# Autodesk Inventor assembly: hip_link2
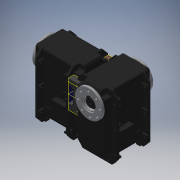
[picture p0: Inventor's stored thumbnail of the model, 180x180]
Saved by Autodesk Inventor 2018 (Build 220112000, 112)
## iProperties
Created: 2018-11-28
Part Number: hip_link2
Document SubType Name: Assembly
Designer: bitbots
Author: bitbots
## Documents named in this file (4)
- C:\Users\bitbots\Desktop\bitbots_hardware\wolfgang\assembly\legs\hip_link2.iam
- C:\Users\bitbots\Desktop\bitbots_hardware\wolfgang\assembly\motors\MX106\MX-106_with_bearing_MIR.iam
- C:\Users\bitbots\Desktop\bitbots_hardware\wolfgang\assembly\legs\motor_connector_MIR.ipt
- C:\Users\bitbots\Desktop\bitbots_hardware\wolfgang\assembly\motors\MX106\MX-106_with_horn_MIR.iam
## Components (4 placed, 3 different names)
1. MX-106_with_bearing_MIR:1 [sub-assembly]
2. motor_connector_MIR:1
3. motor_connector_MIR:2
4. MX-106_with_horn_MIR:1 [sub-assembly] — Mate:10, Mate:11, Angle:1
## Relationships (12: Mate 11, Angle 1)
- [Mate]: MX-106_with_bearing_MIR:1 ↔ motor_connector_MIR:1
- [Mate]: MX-106_with_bearing_MIR:1 ↔ motor_connector_MIR:1
- [Mate]: MX-106_with_bearing_MIR:1 ↔ motor_connector_MIR:1
- [Mate]: MX-106_with_bearing_MIR:1 ↔ motor_connector_MIR:2
- [Mate]: MX-106_with_bearing_MIR:1 ↔ motor_connector_MIR:2
- [Mate]: MX-106_with_bearing_MIR:1 ↔ motor_connector_MIR:2
- [Mate]: motor_connector_MIR:2 ↔ MX-106_with_horn_MIR:1
- [Mate]: motor_connector_MIR:1 ↔ MX-106_with_horn_MIR:1
- [Mate]: motor_connector_MIR:1 ↔ MX-106_with_horn_MIR:1
- Mate:10: MX-106_with_horn_MIR:1
- Mate:11: MX-106_with_horn_MIR:1
- Angle:1 (0 deg): MX-106_with_horn_MIR:1
